# Autodesk Inventor assembly: POM_T5_26
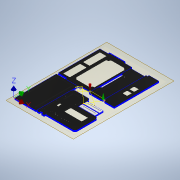
[picture p0: Inventor's stored thumbnail of the model, 180x180]
Saved by Autodesk Inventor 2020 (Build 240168000, 168)
## iProperties
Created: 2021-08-27
Part Number: POM_T5_26
Document SubType Name: Assembly
Designer: Masato
Author: Masato
## Documents named in this file (8)
- C:\Users\ptcga\OneDrive\ドキュメント\SUSTAINA-OP\Cam\POM_T5_26.iam
- C:\Users\ptcga\OneDrive\ドキュメント\SUSTAINA-OP\Cam\DisposableBoard.ipt
- C:\Users\ptcga\OneDrive\ドキュメント\SUSTAINA-OP\UpperBody\Cockpit\Cockpit_circuit_board_frame.ipt
- C:\Users\ptcga\OneDrive\ドキュメント\SUSTAINA-OP\UpperBody\Cockpit\Cockpit_battery_back_door.ipt
- C:\Users\ptcga\OneDrive\ドキュメント\SUSTAINA-OP\UpperBody\Cockpit\Cockpit_top_frame.ipt
- C:\Users\ptcga\OneDrive\ドキュメント\SUSTAINA-OP\UpperBody\Cockpit\Cockpit_front_frame.ipt
- C:\Users\ptcga\OneDrive\ドキュメント\SUSTAINA-OP\UpperBody\Cockpit\Cockpit_side_frame.ipt
- C:\Users\ptcga\OneDrive\ドキュメント\SUSTAINA-OP\Jig\FrontLink_diagonal_Jig.ipt
## Components (8 placed, 7 different names)
1. DisposableBoard:1 — メイト:2, メイト:1, フラッシュ:1, フラッシュ:2, メイト:21, メイト:22, メイト:24, メイト:28, フラッシュ:7, フラッシュ:8, メイト:36, メイト:38
2. Cockpit_circuit_board_frame:1 — メイト:28, メイト:34, フラッシュ:9, フラッシュ:10
3. Cockpit_battery_back_door:1 — メイト:21, フラッシュ:6, メイト:34, メイト:35, フラッシュ:10
4. Cockpit_top_frame:1 — メイト:22, メイト:27, フラッシュ:6, メイト:35
5. Cockpit_front_frame:1 — メイト:24, メイト:27, フラッシュ:7, フラッシュ:8, フラッシュ:9, フラッシュ:11, メイト:37
6. Cockpit_side_frame:1 — メイト:36, フラッシュ:11, メイト:37, メイト:39, メイト:40
7. FrontLink_diagonal_Jig:1 — メイト:38, メイト:39, メイト:40
8. FrontLink_diagonal_Jig:2
## Component patterns: (2 elements, first: FrontLink_diagonal_Jig:1)
## Relationships (22: Mate 14, Flush 8)
- メイト:2 [Mate]: DisposableBoard:1
- メイト:1 [Mate]: DisposableBoard:1
- フラッシュ:1 [Flush]: DisposableBoard:1
- フラッシュ:2 [Flush]: DisposableBoard:1
- メイト:21 [Mate]: DisposableBoard:1 ↔ Cockpit_battery_back_door:1
- メイト:22 [Mate]: DisposableBoard:1 ↔ Cockpit_top_frame:1
- メイト:24 [Mate]: DisposableBoard:1 ↔ Cockpit_front_frame:1
- メイト:27 [Mate] (2.5 mm): Cockpit_top_frame:1 ↔ Cockpit_front_frame:1
- フラッシュ:6 [Flush]: Cockpit_battery_back_door:1 ↔ Cockpit_top_frame:1
- メイト:28 [Mate]: DisposableBoard:1 ↔ Cockpit_circuit_board_frame:1
- メイト:34 [Mate] (2.5 mm): Cockpit_circuit_board_frame:1 ↔ Cockpit_battery_back_door:1
- メイト:35 [Mate] (2.5 mm): Cockpit_battery_back_door:1 ↔ Cockpit_top_frame:1
- フラッシュ:7 [Flush] (2.5 mm): DisposableBoard:1 ↔ Cockpit_front_frame:1
- フラッシュ:8 [Flush] (2.5 mm): DisposableBoard:1 ↔ Cockpit_front_frame:1
- フラッシュ:9 [Flush]: Cockpit_circuit_board_frame:1 ↔ Cockpit_front_frame:1
- フラッシュ:10 [Flush]: Cockpit_circuit_board_frame:1 ↔ Cockpit_battery_back_door:1
- メイト:36 [Mate]: DisposableBoard:1 ↔ Cockpit_side_frame:1
- フラッシュ:11 [Flush]: Cockpit_front_frame:1 ↔ Cockpit_side_frame:1
- メイト:37 [Mate] (2.5 mm): Cockpit_front_frame:1 ↔ Cockpit_side_frame:1
- メイト:38 [Mate]: DisposableBoard:1 ↔ FrontLink_diagonal_Jig:1
- メイト:39 [Mate] (2.5 mm): Cockpit_side_frame:1 ↔ FrontLink_diagonal_Jig:1
- メイト:40 [Mate] (2.5 mm): Cockpit_side_frame:1 ↔ FrontLink_diagonal_Jig:1
